# Autodesk Inventor assembly: bloc_double106_MIR
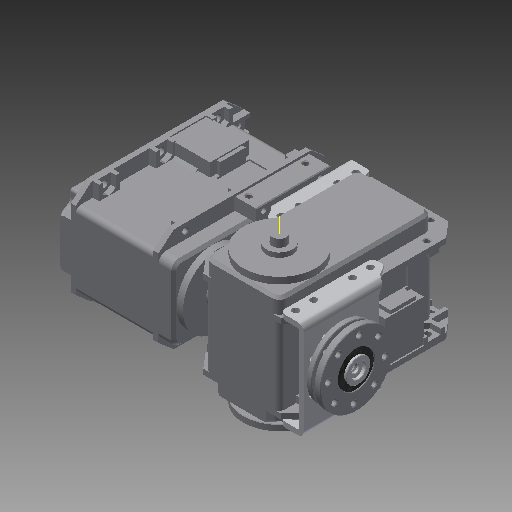
[picture p0: Inventor's stored thumbnail of the model, 512x512]
Saved by Autodesk Inventor 2018 (Build 220112000, 112)
## iProperties
Created: 2017-02-17
Part Number: bloc_double106_MIR
Document SubType Name: Assembly
Designer: steve
Mass: 340.305 g
Surface Area: 512.023 cm^2
Volume: 186.598 cm^3
Density: 1.82373 g/cm^3
Author: steve
## Documents named in this file (8)
- C:\Users\medrimonia\Dropbox\SigmaBan\SigmaBanV2.1\bloc_double106_MIR.iam
- C:\Users\medrimonia\Dropbox\SigmaBan\SigmaBanV2.1\MX-106T.ipt
- C:\Users\medrimonia\Dropbox\SigmaBan\SigmaBanV2.1\RX64-CAP.ipt
- C:\Users\medrimonia\Dropbox\SigmaBan\SigmaBanV2.1\MF128ZZ.ipt
- C:\Users\medrimonia\Dropbox\SigmaBan\SigmaBanV2.1\dynamixel\frames\FR08-B101.ipt
- C:\Users\medrimonia\Dropbox\SigmaBan\SigmaBanV2.1\FR05-S101.ipt
- C:\Users\medrimonia\Dropbox\SigmaBan\SigmaBanV2.1\dynamixel\horn\HN05-i101.ipt
- C:\Users\medrimonia\Dropbox\SigmaBan\SigmaBanV2.1\dynamixel\frames\FR05-F101.ipt
## Components (12 placed, 7 different names)
1. MX-106T:1 — Mate:8, Mate:26, Mate:27, Mate:30, Mate:40, Mate:41, Mate:42, Mate:44, Mate:45, Mate:46, Flush:2, Mate:56
2. MX-106T:2 — Mate:13, Mate:31, Mate:35, Mate:36, Mate:37, Mate:50, Mate:59
3. RX64-CAP:1 — Mate:26
4. MF128ZZ:1 — Mate:27
5. FR08-B101:1 — Mate:35, Mate:36, Mate:37, Mate:47, Mate:48
6. FR05-S101:1 — Mate:40, Mate:41, Mate:42, Mate:51, Mate:52
7. FR05-S101:2 — Mate:44, Mate:45, Mate:46, Mate:47, Mate:48
8. HN05-i101:2 — Mate:50, Mate:57
9. FR05-F101:1 — Mate:51, Mate:52, Mate:53, Mate:54
10. RX64-CAP:2 — Mate:53, Mate:54, Mate:58
11. HN05-i101:3 — Flush:2, Mate:56
12. MF128ZZ:2 — Mate:57, Mate:58, Mate:59
## Relationships (29: Mate 28, Flush 1)
- Mate:8: MX-106T:1
- Mate:13: MX-106T:2
- [Mate]: RX64-CAP:1 ↔ MF128ZZ:1
- [Mate]: RX64-CAP:1 ↔ MF128ZZ:1
- Mate:26: MX-106T:1 ↔ RX64-CAP:1
- Mate:27: MX-106T:1 ↔ MF128ZZ:1
- Mate:30: MX-106T:1
- Mate:31: MX-106T:2
- Mate:35: MX-106T:2 ↔ FR08-B101:1
- Mate:36: MX-106T:2 ↔ FR08-B101:1
- Mate:37: MX-106T:2 ↔ FR08-B101:1
- Mate:40: MX-106T:1 ↔ FR05-S101:1
- Mate:41: MX-106T:1 ↔ FR05-S101:1
- Mate:42: MX-106T:1 ↔ FR05-S101:1
- Mate:44: MX-106T:1 ↔ FR05-S101:2
- Mate:45: MX-106T:1 ↔ FR05-S101:2
- Mate:46: MX-106T:1 ↔ FR05-S101:2
- Mate:47: FR08-B101:1 ↔ FR05-S101:2
- Mate:48: FR08-B101:1 ↔ FR05-S101:2
- Mate:50: MX-106T:2 ↔ HN05-i101:2
- Mate:51: FR05-S101:1 ↔ FR05-F101:1
- Mate:52: FR05-S101:1 ↔ FR05-F101:1
- Mate:53: FR05-F101:1 ↔ RX64-CAP:2
- Mate:54: FR05-F101:1 ↔ RX64-CAP:2
- Flush:2 (-3 mm): MX-106T:1 ↔ HN05-i101:3
- Mate:56: MX-106T:1 ↔ HN05-i101:3
- Mate:57: HN05-i101:2 ↔ MF128ZZ:2
- Mate:58: RX64-CAP:2 ↔ MF128ZZ:2
- Mate:59: MX-106T:2 ↔ MF128ZZ:2
## Named parameters: d29_d27 = 0 mm
